# Autodesk Inventor assembly: fullbody
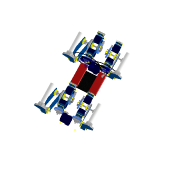
[picture p0: Inventor's stored thumbnail of the model, 180x180]
Saved by Autodesk Inventor 2020.5 (Build 245400000, 400)
## iProperties
Created: 2022-11-17
Part Number: fullbody
Document SubType Name: Assembly
Designer: kanazawakotaro
Author: kanazawakotaro
## Documents named in this file (7)
- C:\Users\Administrator\Documents\kamuy2\kamuy2\fullbody.iam
- C:\Users\Administrator\Documents\kamuy2\kamuy2\VER2.0_MIR_CPY.iam
- C:\Users\Administrator\Documents\kamuy2\kamuy2\VER2.0_MIR_CPY_MIR.iam
- C:\Users\Administrator\Documents\kamuy2\kamuy2\3dprinter\Part1.ipt
- C:\Users\Administrator\Documents\kamuy2\kamuy2\Parts\BGTAB6900VV_Autodesk_Inventor_2020_20221121\AIS2020\BGTAB6900VV.iam
- C:\Users\Administrator\Documents\kamuy2\kamuy2\3dprinter\lipo.ipt
- C:\Users\Administrator\Documents\kamuy2\kamuy2\3dprinter\nuc.ipt
## Components (12 placed, 6 different names)
1. VER2.0_MIR_CPY:1 [sub-assembly] — フラッシュ:14, フラッシュ:15, メイト:1
2. VER2.0_MIR_CPY_MIR:1 [sub-assembly] — フラッシュ:14, フラッシュ:15, メイト:1, フラッシュ:18, フラッシュ:19, フラッシュ:21
3. VER2.0_MIR_CPY:2 [sub-assembly] — フラッシュ:24
4. VER2.0_MIR_CPY_MIR:2 [sub-assembly] — フラッシュ:18, フラッシュ:19, フラッシュ:20
5. Part1:1 — フラッシュ:20
6. BGTAB6900VV:1 [sub-assembly]
7. BGTAB6900VV:2 [sub-assembly]
8. BGTAB6900VV:3 [sub-assembly]
9. BGTAB6900VV:4 [sub-assembly]
10. lipo:1 — フラッシュ:23, フラッシュ:24, フラッシュ:25, フラッシュ:26
11. lipo:2 — フラッシュ:22, フラッシュ:25
12. nuc:1 — フラッシュ:21, フラッシュ:22, フラッシュ:23, フラッシュ:26
## Relationships (15: Flush 13, Mate 2)
- フラッシュ:14 [Flush]: VER2.0_MIR_CPY:1 ↔ VER2.0_MIR_CPY_MIR:1
- フラッシュ:15 [Flush]: VER2.0_MIR_CPY:1 ↔ VER2.0_MIR_CPY_MIR:1
- メイト:1 [Mate]: VER2.0_MIR_CPY:1 ↔ VER2.0_MIR_CPY_MIR:1
- [Flush]: VER2.0_MIR_CPY:2 ↔ VER2.0_MIR_CPY_MIR:2
- [Flush]: VER2.0_MIR_CPY:2 ↔ VER2.0_MIR_CPY_MIR:2
- [Mate]: VER2.0_MIR_CPY:2 ↔ VER2.0_MIR_CPY_MIR:2
- フラッシュ:18 [Flush]: VER2.0_MIR_CPY_MIR:1 ↔ VER2.0_MIR_CPY_MIR:2
- フラッシュ:19 [Flush]: VER2.0_MIR_CPY_MIR:1 ↔ VER2.0_MIR_CPY_MIR:2
- フラッシュ:20 [Flush]: VER2.0_MIR_CPY_MIR:2 ↔ Part1:1
- フラッシュ:21 [Flush] (-50 mm): VER2.0_MIR_CPY_MIR:1 ↔ nuc:1
- フラッシュ:22 [Flush] (50 mm): lipo:2 ↔ nuc:1
- フラッシュ:23 [Flush] (50 mm): lipo:1 ↔ nuc:1
- フラッシュ:24 [Flush] (30 mm): VER2.0_MIR_CPY:2 ↔ lipo:1
- フラッシュ:25 [Flush]: lipo:1 ↔ lipo:2
- フラッシュ:26 [Flush] (20 mm): lipo:1 ↔ nuc:1
## Named parameters: d20_d16 = 0 mm, d21_d18 = 0 mm, d22_d19 = 0 mm
